# Autodesk Inventor assembly: Robot
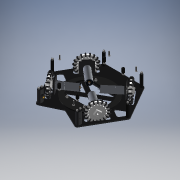
[picture p0: Inventor's stored thumbnail of the model, 180x180]
Saved by Autodesk Inventor 2017 (Build 210142000, 142)
## iProperties
Created: 2016-10-01
Part Number: Robot
Document SubType Name: Assembly
Designer: James Yelland
Author: James Yelland
## Documents named in this file (28)
- C:\Users\yella\git\LJ-STAND\Design\Models\Robot\Robot.iam
- C:\Users\yella\git\LJ-STAND\Design\Models\Robot\Bottom Plate.ipt
- C:\Users\yella\git\LJ-STAND\Design\Models\Robot\Motor Mount.ipt
- C:\Users\yella\git\LJ-STAND\Design\Models\Fasteners\Standoff 30 F-F.ipt
- C:\Users\yella\git\LJ-STAND\Design\Models\Robot\LDR mount.ipt
- C:\Users\yella\git\LJ-STAND\Design\Models\Robot\Laser diode mount.ipt
- C:\Users\yella\git\LJ-STAND\Design\Models\Fasteners\M3x10 Screw.ipt
- C:\Users\yella\git\LJ-STAND\Design\Models\Fasteners\M3 Hex Nut.ipt
- C:\Users\yella\git\LJ-STAND\Design\Models\Common\Imported Components\maxon_PN_0_1\maxon_PN_0_1.iam
- C:\Users\yella\git\LJ-STAND\Design\Models\Fasteners\M2x4 Screw.ipt
- C:\Users\yella\git\LJ-STAND\Design\Models\Robot\Light Sensor PCB.ipt
- C:\Users\yella\git\LJ-STAND\Design\Models\Common\Wheel.ipt
- C:\Users\yella\git\LJ-STAND\Design\Models\Robot\Middle Plate.ipt
- C:\Users\yella\git\LJ-STAND\Design\Models\Fasteners\Standoff 10 M-F.ipt
- C:\Users\yella\git\LJ-STAND\Design\Models\Robot\TSOP Cover Ring.ipt
- C:\Users\yella\git\LJ-STAND\Design\Models\Robot\Main PCB.ipt
- C:\Users\yella\git\LJ-STAND\Design\Models\Fasteners\M3x20 Screw.ipt
- C:\Users\yella\git\LJ-STAND\Design\Models\Common\Laser Diode.ipt
- C:\Users\yella\git\LJ-STAND\Design\Models\Common\Pixy angle bracket.ipt
- C:\Users\yella\git\LJ-STAND\Design\Models\Pixy\pixy\Imported Components\Pixy(CMUcam5)\Pixy(CMUcam5).iam
- C:\Users\yella\git\LJ-STAND\Design\Models\Fasteners\Standoff 65 M-F.ipt
- C:\Users\yella\git\LJ-STAND\Design\Models\Robot\Top Plate.ipt
- C:\Users\yella\git\LJ-STAND\Design\Models\Robot\Handle.ipt
- C:\Users\yella\git\LJ-STAND\Design\Models\Common\Rocker switch.ipt
- C:\Users\yella\git\LJ-STAND\Design\Models\Fasteners\Standoff 25 F-F.ipt
- C:\Users\yella\git\LJ-STAND\Design\Models\Robot\Sonar Mount.ipt
- C:\Users\yella\git\LJ-STAND\Design\Models\Fasteners\M3x6 Screw.ipt
- C:\Users\yella\git\LJ-STAND\Design\Models\Common\Sonar.ipt
## Components (119 placed, 27 different names)
1. Bottom Plate:1 — Insert:1, Insert:2, Insert:3, Insert:4, Insert:5, Insert:6, Insert:7, Insert:8, Insert:31, Insert:32, Insert:33, Insert:34, Insert:35, Insert:36, Insert:37, Insert:38, Insert:39, Insert:40, Insert:45, Insert:46, Insert:47, Insert:48, Mate:27, Mate:28, Mate:29, Mate:30, Mate:31, Mate:32, Mate:33, Mate:34, Mate:35, Mate:36, Mate:37, Mate:38
2. Motor Mount:1 — Insert:15, Mate:13, Insert:25, Insert:26, Insert:27, Mate:33, Mate:34, Mate:35
3. Motor Mount:2 — Insert:16, Mate:14, Insert:22, Insert:23, Insert:24, Mate:27, Mate:28, Mate:29
4. Motor Mount:3 — Insert:18, Mate:15, Insert:19, Insert:20, Insert:21, Mate:36, Mate:37, Mate:38
5. Motor Mount:4 — Insert:17, Mate:16, Insert:28, Insert:29, Insert:30, Mate:30, Mate:31, Mate:32
6. Standoff 30 F-F:1 — Insert:3
7. Standoff 30 F-F:2 — Insert:4
8. Standoff 30 F-F:3 — Insert:2, Insert:50, Insert:127
9. Standoff 30 F-F:4 — Insert:1, Insert:49, Insert:126
10. LDR mount:1 — Insert:33, Insert:34
11. Laser diode mount:1 — Insert:31, Insert:32, Insert:93
12. M3x10 Screw:1 — Insert:5
13. M3x10 Screw:2 — Insert:7
14. M3x10 Screw:3 — Insert:6
15. M3x10 Screw:4 — Insert:8
16. maxon_PN_0_1:1 [sub-assembly] — Insert:16, Mate:14, Mate:18, Flush:2
17. maxon_PN_0_1:2 [sub-assembly] — Insert:17, Mate:16, Mate:20, Flush:4
18. maxon_PN_0_1:3 [sub-assembly] — Insert:15, Mate:13, Mate:19, Flush:3
19. maxon_PN_0_1:4 [sub-assembly] — Insert:18, Mate:15, Mate:17, Flush:1
20. M2x4 Screw:1 — Insert:25
21. M2x4 Screw:3 — Insert:19
22. M2x4 Screw:4 — Insert:28
23. M2x4 Screw:5 — Insert:27
24. M2x4 Screw:6 — Insert:26
25. M2x4 Screw:7 — Insert:24
26. M2x4 Screw:8 — Insert:21
27. M2x4 Screw:9 — Insert:20
28. M2x4 Screw:10 — Insert:29
29. M2x4 Screw:11 — Insert:23
30. M2x4 Screw:12 — Insert:22
31. M2x4 Screw:13 — Insert:30
32. Light Sensor PCB:1 — Insert:35, Insert:36, Insert:41, Insert:42, Insert:43, Insert:44
33. M3 Hex Nut:3 — Insert:41
34. M3x10 Screw:7 — Insert:37
35. M3 Hex Nut:4 — Insert:42
36. M3x10 Screw:8 — Insert:38
37. M3 Hex Nut:5 — Insert:43
38. M3x10 Screw:9 — Insert:39
39. M3 Hex Nut:6 — Insert:44
40. M3x10 Screw:10 — Insert:40
41. M3x10 Screw:11 — Insert:45
42. M3x10 Screw:12 — Insert:46
43. M3x10 Screw:13 — Insert:47
44. M3x10 Screw:14 — Insert:48
45. Wheel:1 — Mate:18, Flush:2
46. Wheel:2 — Mate:19, Flush:3
47. Wheel:3 — Mate:17, Flush:1
48. Wheel:4 — Mate:20, Flush:4
49. Middle Plate:1 — Insert:49, Insert:50, Insert:51, Insert:52, Insert:53, Insert:54, Insert:59, Insert:60, Insert:61, Insert:62, Insert:63, Insert:64, Insert:65, Insert:66, Insert:102, Insert:103, Insert:104, Insert:105, Insert:106, Insert:107, Insert:120, Insert:121, Insert:122, Insert:123, Insert:124, Insert:125, Insert:126, Insert:127, Insert:128, Insert:129, Insert:130, Insert:131
50. M3x10 Screw:15 — Insert:51
51. M3x10 Screw:16 — Insert:52
52. M3x10 Screw:17 — Insert:53
53. M3x10 Screw:18 — Insert:54
54. Standoff 10 M-F:1 — Insert:59
55. Standoff 10 M-F:2 — Insert:60
56. Standoff 10 M-F:3 — Insert:61, Insert:67
57. Standoff 10 M-F:4 — Insert:62, Insert:68
58. M3 Hex Nut:11 — Insert:65
59. M3 Hex Nut:12 — Insert:66
60. M3 Hex Nut:13 — Insert:64
61. M3 Hex Nut:14 — Insert:63
62. TSOP Cover Ring:1 — Insert:67, Insert:68, Insert:69, Insert:70, Angle:1, Angle:2
63. Main PCB:1 — Insert:69, Insert:70, Insert:71, Insert:72, Insert:73, Insert:74, Insert:94, Insert:95
64. M3x20 Screw:1 — Insert:74
65. M3x20 Screw:2 — Insert:73
66. M3x20 Screw:3 — Insert:72
67. M3x20 Screw:4 — Insert:71
68. Laser Diode:1 — Insert:93
69. Pixy angle bracket:1 — Insert:95, Angle:2, Insert:168
70. Pixy angle bracket:2 — Insert:94, Angle:1, Insert:169
71. Pixy(CMUcam5):1 [sub-assembly] — Insert:168, Insert:169
72. Standoff 65 M-F:3 — Insert:102
73. Standoff 65 M-F:4 — Insert:103, Insert:140
74. Standoff 65 M-F:5 — Insert:106
75. Standoff 65 M-F:6 — Insert:107
76. Standoff 65 M-F:7 — Insert:105, Insert:141
77. Standoff 65 M-F:8 — Insert:104
78. Handle:1 — Insert:136, Insert:137, Insert:138, Insert:139
79. M3x10 Screw:19 — Insert:120
80. M3x10 Screw:20 — Insert:122
81. M3 Hex Nut:17 — Insert:146
82. M3x10 Screw:21 — Insert:125
83. M3 Hex Nut:18 — Insert:144
84. M3x10 Screw:22 — Insert:124
85. M3 Hex Nut:19 — Insert:151
86. M3x10 Screw:23 — Insert:123
87. M3 Hex Nut:20 — Insert:150
88. M3x10 Screw:24 — Insert:121
89. Rocker switch:1 — Mate:21, Mate:22, Mate:23
90. Rocker switch:2 — Mate:24, Mate:25, Mate:26
91. M3x10 Screw:25 — Insert:131
92. M3x10 Screw:26 — Insert:130
93. M3x10 Screw:27 — Insert:129
94. M3x10 Screw:28 — Insert:128
95. Standoff 25 F-F:1 — Insert:137, Insert:143
96. Standoff 25 F-F:2 — Insert:136, Insert:142
97. M3x10 Screw:29 — Insert:149
98. M3x10 Screw:30 — Insert:145
99. M3x10 Screw:31 — Insert:139
100. M3x10 Screw:32 — Insert:138
101. M3 Hex Nut:21 — Insert:147
102. M3 Hex Nut:22 — Insert:148
103. Sonar Mount:1 — Insert:156, Insert:157, Insert:170, Insert:171
104. Sonar Mount:2 — Insert:158, Insert:159, Insert:172, Insert:173
105. Sonar Mount:3 — Insert:152, Insert:153, Insert:176, Insert:177
106. Sonar Mount:4 — Insert:154, Insert:155, Insert:174, Insert:175
107. Top Plate:1 — Insert:140, Insert:141, Insert:142, Insert:143, Insert:144, Insert:145, Insert:146, Insert:147, Insert:148, Insert:149, Insert:150, Insert:151, Insert:152, Insert:153, Insert:154, Insert:155, Mate:21, Mate:22, Mate:23, Mate:24, Mate:25, Mate:26, Insert:156, Insert:157, Insert:158, Insert:159, Insert:160, Insert:161, Insert:162, Insert:163, Insert:164, Insert:165, Insert:166, Insert:167
108. M3x6 Screw:1 — Insert:160
109. M3x6 Screw:2 — Insert:161
110. M3x6 Screw:3 — Insert:162
111. M3x6 Screw:4 — Insert:167
112. M3x6 Screw:5 — Insert:163
113. M3x6 Screw:6 — Insert:165
114. M3x6 Screw:7 — Insert:166
115. M3x6 Screw:8 — Insert:164
116. Sonar:1 — Insert:176, Insert:177
117. Sonar:2 — Insert:174, Insert:175
118. Sonar:3 — Insert:172, Insert:173
119. Sonar:4 — Insert:170, Insert:171
## Relationships (159: Insert 127, Mate 26, Flush 4, Angle 2)
- Insert:1: Bottom Plate:1 ↔ Standoff 30 F-F:4
- Insert:2: Bottom Plate:1 ↔ Standoff 30 F-F:3
- Insert:3: Bottom Plate:1 ↔ Standoff 30 F-F:1
- Insert:4: Bottom Plate:1 ↔ Standoff 30 F-F:2
- Insert:5: Bottom Plate:1 ↔ M3x10 Screw:1
- Insert:6: Bottom Plate:1 ↔ M3x10 Screw:3
- Insert:7: Bottom Plate:1 ↔ M3x10 Screw:2
- Insert:8: Bottom Plate:1 ↔ M3x10 Screw:4
- Insert:15: Motor Mount:1 ↔ maxon_PN_0_1:3
- Insert:16: Motor Mount:2 ↔ maxon_PN_0_1:1
- Insert:17: Motor Mount:4 ↔ maxon_PN_0_1:2
- Insert:18: Motor Mount:3 ↔ maxon_PN_0_1:4
- Mate:13: Motor Mount:1 ↔ maxon_PN_0_1:3
- Mate:14: Motor Mount:2 ↔ maxon_PN_0_1:1
- Mate:15: Motor Mount:3 ↔ maxon_PN_0_1:4
- Mate:16: Motor Mount:4 ↔ maxon_PN_0_1:2
- Insert:19: Motor Mount:3 ↔ M2x4 Screw:3
- Insert:20: Motor Mount:3 ↔ M2x4 Screw:9
- Insert:21: Motor Mount:3 ↔ M2x4 Screw:8
- Insert:22: Motor Mount:2 ↔ M2x4 Screw:12
- Insert:23: Motor Mount:2 ↔ M2x4 Screw:11
- Insert:24: Motor Mount:2 ↔ M2x4 Screw:7
- Insert:25: Motor Mount:1 ↔ M2x4 Screw:1
- Insert:26: Motor Mount:1 ↔ M2x4 Screw:6
- Insert:27: Motor Mount:1 ↔ M2x4 Screw:5
- Insert:28: Motor Mount:4 ↔ M2x4 Screw:4
- Insert:29: Motor Mount:4 ↔ M2x4 Screw:10
- Insert:30: Motor Mount:4 ↔ M2x4 Screw:13
- Insert:31: Bottom Plate:1 ↔ Laser diode mount:1
- Insert:32: Bottom Plate:1 ↔ Laser diode mount:1
- Insert:33: Bottom Plate:1 ↔ LDR mount:1
- Insert:34: Bottom Plate:1 ↔ LDR mount:1
- Insert:35: Bottom Plate:1 ↔ Light Sensor PCB:1
- Insert:36: Bottom Plate:1 ↔ Light Sensor PCB:1
- Insert:37: Bottom Plate:1 ↔ M3x10 Screw:7
- Insert:38: Bottom Plate:1 ↔ M3x10 Screw:8
- Insert:39: Bottom Plate:1 ↔ M3x10 Screw:9
- Insert:40: Bottom Plate:1 ↔ M3x10 Screw:10
- Insert:41: Light Sensor PCB:1 ↔ M3 Hex Nut:3
- Insert:42: Light Sensor PCB:1 ↔ M3 Hex Nut:4
- Insert:43: Light Sensor PCB:1 ↔ M3 Hex Nut:5
- Insert:44: Light Sensor PCB:1 ↔ M3 Hex Nut:6
- Insert:45: Bottom Plate:1 ↔ M3x10 Screw:11
- Insert:46: Bottom Plate:1 ↔ M3x10 Screw:12
- Insert:47: Bottom Plate:1 ↔ M3x10 Screw:13
- Insert:48: Bottom Plate:1 ↔ M3x10 Screw:14
- Mate:17: maxon_PN_0_1:4 ↔ Wheel:3
- Flush:1 (-7 mm): maxon_PN_0_1:4 ↔ Wheel:3
- Mate:18: maxon_PN_0_1:1 ↔ Wheel:1
- Flush:2 (-7 mm): maxon_PN_0_1:1 ↔ Wheel:1
- Mate:19: maxon_PN_0_1:3 ↔ Wheel:2
- Flush:3 (-7 mm): maxon_PN_0_1:3 ↔ Wheel:2
- Mate:20: maxon_PN_0_1:2 ↔ Wheel:4
- Flush:4 (-7 mm): maxon_PN_0_1:2 ↔ Wheel:4
- Insert:49: Standoff 30 F-F:4 ↔ Middle Plate:1
- Insert:50: Standoff 30 F-F:3 ↔ Middle Plate:1
- Insert:51: Middle Plate:1 ↔ M3x10 Screw:15
- Insert:52: Middle Plate:1 ↔ M3x10 Screw:16
- Insert:53: Middle Plate:1 ↔ M3x10 Screw:17
- Insert:54: Middle Plate:1 ↔ M3x10 Screw:18
- Insert:59: Middle Plate:1 ↔ Standoff 10 M-F:1
- Insert:60: Middle Plate:1 ↔ Standoff 10 M-F:2
- Insert:61: Middle Plate:1 ↔ Standoff 10 M-F:3
- Insert:62: Middle Plate:1 ↔ Standoff 10 M-F:4
- Insert:63: Middle Plate:1 ↔ M3 Hex Nut:14
- Insert:64: Middle Plate:1 ↔ M3 Hex Nut:13
- Insert:65: Middle Plate:1 ↔ M3 Hex Nut:11
- Insert:66: Middle Plate:1 ↔ M3 Hex Nut:12
- Insert:67: Standoff 10 M-F:3 ↔ TSOP Cover Ring:1
- Insert:68: Standoff 10 M-F:4 ↔ TSOP Cover Ring:1
- Insert:69: TSOP Cover Ring:1 ↔ Main PCB:1
- Insert:70: TSOP Cover Ring:1 ↔ Main PCB:1
- Insert:71: Main PCB:1 ↔ M3x20 Screw:4
- Insert:72: Main PCB:1 ↔ M3x20 Screw:3
- Insert:73: Main PCB:1 ↔ M3x20 Screw:2
- Insert:74: Main PCB:1 ↔ M3x20 Screw:1
- Insert:93: Laser diode mount:1 ↔ Laser Diode:1
- Insert:94: Main PCB:1 ↔ Pixy angle bracket:2
- Insert:95: Main PCB:1 ↔ Pixy angle bracket:1
- Insert:102: Middle Plate:1 ↔ Standoff 65 M-F:3
- Insert:103: Middle Plate:1 ↔ Standoff 65 M-F:4
- Insert:104: Middle Plate:1 ↔ Standoff 65 M-F:8
- Insert:105: Middle Plate:1 ↔ Standoff 65 M-F:7
- Insert:106: Middle Plate:1 ↔ Standoff 65 M-F:5
- Insert:107: Middle Plate:1 ↔ Standoff 65 M-F:6
- Insert:120: Middle Plate:1 ↔ M3x10 Screw:19
- Insert:121: Middle Plate:1 ↔ M3x10 Screw:24
- Insert:122: Middle Plate:1 ↔ M3x10 Screw:20
- Insert:123: Middle Plate:1 ↔ M3x10 Screw:23
- Insert:124: Middle Plate:1 ↔ M3x10 Screw:22
- Insert:125: Middle Plate:1 ↔ M3x10 Screw:21
- Insert:126: Standoff 30 F-F:4 ↔ Middle Plate:1
- Insert:127: Standoff 30 F-F:3 ↔ Middle Plate:1
- Insert:128: Middle Plate:1 ↔ M3x10 Screw:28
- Insert:129: Middle Plate:1 ↔ M3x10 Screw:27
- Insert:130: Middle Plate:1 ↔ M3x10 Screw:26
- Insert:131: Middle Plate:1 ↔ M3x10 Screw:25
- Insert:136: Handle:1 ↔ Standoff 25 F-F:2
- Insert:137: Handle:1 ↔ Standoff 25 F-F:1
- Insert:138: Handle:1 ↔ M3x10 Screw:32
- Insert:139: Handle:1 ↔ M3x10 Screw:31
- Insert:140: Standoff 65 M-F:4 ↔ Top Plate:1
- Insert:141: Standoff 65 M-F:7 ↔ Top Plate:1
- Insert:142: Standoff 25 F-F:2 ↔ Top Plate:1
- Insert:143: Standoff 25 F-F:1 ↔ Top Plate:1
- Insert:144: M3 Hex Nut:18 ↔ Top Plate:1
- Insert:145: M3x10 Screw:30 ↔ Top Plate:1
- Insert:146: M3 Hex Nut:17 ↔ Top Plate:1
- Insert:147: M3 Hex Nut:21 ↔ Top Plate:1
- Insert:148: M3 Hex Nut:22 ↔ Top Plate:1
- Insert:149: M3x10 Screw:29 ↔ Top Plate:1
- Insert:150: M3 Hex Nut:20 ↔ Top Plate:1
- Insert:151: M3 Hex Nut:19 ↔ Top Plate:1
- Insert:152: Sonar Mount:3 ↔ Top Plate:1
- Insert:153: Sonar Mount:3 ↔ Top Plate:1
- Insert:154: Sonar Mount:4 ↔ Top Plate:1
- Insert:155: Sonar Mount:4 ↔ Top Plate:1
- Mate:21: Rocker switch:1 ↔ Top Plate:1
- Mate:22: Rocker switch:1 ↔ Top Plate:1
- Mate:23: Rocker switch:1 ↔ Top Plate:1
- Mate:24: Rocker switch:2 ↔ Top Plate:1
- Mate:25: Rocker switch:2 ↔ Top Plate:1
- Mate:26: Rocker switch:2 ↔ Top Plate:1
- Insert:156: Sonar Mount:1 ↔ Top Plate:1
- Insert:157: Sonar Mount:1 ↔ Top Plate:1
- Insert:158: Sonar Mount:2 ↔ Top Plate:1
- Insert:159: Sonar Mount:2 ↔ Top Plate:1
- Insert:160: Top Plate:1 ↔ M3x6 Screw:1
- Insert:161: Top Plate:1 ↔ M3x6 Screw:2
- Insert:162: Top Plate:1 ↔ M3x6 Screw:3
- Insert:163: Top Plate:1 ↔ M3x6 Screw:5
- Insert:164: Top Plate:1 ↔ M3x6 Screw:8
- Insert:165: Top Plate:1 ↔ M3x6 Screw:6
- Insert:166: Top Plate:1 ↔ M3x6 Screw:7
- Insert:167: Top Plate:1 ↔ M3x6 Screw:4
- Angle:1 (0 deg): TSOP Cover Ring:1 ↔ Pixy angle bracket:2
- Angle:2 (0 deg): TSOP Cover Ring:1 ↔ Pixy angle bracket:1
- Insert:168: Pixy angle bracket:1 ↔ Pixy(CMUcam5):1
- Insert:169: Pixy angle bracket:2 ↔ Pixy(CMUcam5):1
- Insert:170: Sonar Mount:1 ↔ Sonar:4
- Insert:171: Sonar Mount:1 ↔ Sonar:4
- Insert:172: Sonar Mount:2 ↔ Sonar:3
- Insert:173: Sonar Mount:2 ↔ Sonar:3
- Insert:174: Sonar Mount:4 ↔ Sonar:2
- Insert:175: Sonar Mount:4 ↔ Sonar:2
- Insert:176: Sonar Mount:3 ↔ Sonar:1
- Insert:177: Sonar Mount:3 ↔ Sonar:1
- Mate:27: Bottom Plate:1 ↔ Motor Mount:2
- Mate:28: Bottom Plate:1 ↔ Motor Mount:2
- Mate:29: Bottom Plate:1 ↔ Motor Mount:2
- Mate:30: Bottom Plate:1 ↔ Motor Mount:4
- Mate:31: Bottom Plate:1 ↔ Motor Mount:4
- Mate:32: Bottom Plate:1 ↔ Motor Mount:4
- Mate:33: Bottom Plate:1 ↔ Motor Mount:1
- Mate:34: Bottom Plate:1 ↔ Motor Mount:1
- Mate:35: Bottom Plate:1 ↔ Motor Mount:1
- Mate:36: Bottom Plate:1 ↔ Motor Mount:3
- Mate:37: Bottom Plate:1 ↔ Motor Mount:3
- Mate:38: Bottom Plate:1 ↔ Motor Mount:3
